# Autodesk Inventor assembly: Soporte placa
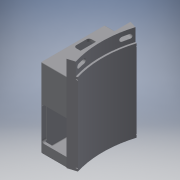
[picture p0: Inventor's stored thumbnail of the model, 180x180]
Saved by Autodesk Inventor 2019 (Build 230136000, 136)
## iProperties
Created: 2020-08-10
Part Number: Soporte placa
Document SubType Name: Assembly
Designer: Hugo Albarracin
Author: Hugo Albarracin
## Documents named in this file (4)
- C:\Users\Hugo Albarracin\OneDrive - Escuela Superior Politécnica del Litoral\U - UPM ELECTROMECANICA\14. TFM\iris_mecanico\Soporte placa.iam
- C:\Users\Hugo Albarracin\OneDrive - Escuela Superior Politécnica del Litoral\U - UPM ELECTROMECANICA\14. TFM\iris_mecanico\soporte_placa.ipt
- C:\Users\Hugo Albarracin\OneDrive - Escuela Superior Politécnica del Litoral\U - UPM ELECTROMECANICA\14. TFM\iris_mecanico\soporte_placa_techo.ipt
- C:\Users\Hugo Albarracin\OneDrive - Escuela Superior Politécnica del Litoral\U - UPM ELECTROMECANICA\14. TFM\iris_mecanico\soporte_placa_separador.ipt
## Components (3 placed, 3 different names)
1. soporte_placa:1 — Flush:1, Flush:2, Flush:3, Mate:1, Flush:4, Mate:3
2. soporte_placa_techo:1 — Mate:1, Mate:2, Flush:4
3. soporte_placa_separador:1 — Mate:3, Mate:4
## Relationships (8: Flush 4, Mate 4)
- Flush:1: soporte_placa:1
- Flush:2: soporte_placa:1
- Flush:3: soporte_placa:1
- Mate:1: soporte_placa:1 ↔ soporte_placa_techo:1
- Mate:2: soporte_placa_techo:1
- Flush:4: soporte_placa:1 ↔ soporte_placa_techo:1
- Mate:3: soporte_placa:1 ↔ soporte_placa_separador:1
- Mate:4: soporte_placa_separador:1
